# Autodesk Inventor assembly: 76607c01
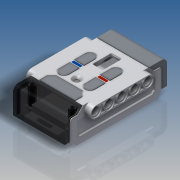
[picture p0: Inventor's stored thumbnail of the model, 180x180]
Saved by Autodesk Inventor 2016 SP2 (Build 200236200, 236)
## iProperties
Created: 2015-08-26
Part Number: 76607c01
Document SubType Name: Assembly
Designer: D. Kohfeld
Mass: 14.5113 g
Surface Area: 211.449 cm^2
Volume: 12.6712 cm^3
Density: 1.14522 g/cm^3
Author: D. Kohfeld
## Documents named in this file (8)
- A:\LEGO Pieces\EV3\76607c01.iam
- A:\LEGO Pieces\EV3\76607p01-White.ipt
- A:\LEGO Pieces\EV3\11235-TransBlackIRLens.ipt
- A:\LEGO Pieces\EV3\11235-LtBluishGray.ipt
- A:\LEGO Pieces\EV3\76608-White.ipt
- A:\LEGO Pieces\EV3\11236-LtBluishGray.ipt
- A:\LEGO Pieces\EV3\76610-LtBluishGray.ipt
- A:\LEGO Pieces\EV3\u9013-Black.ipt
## Components (13 placed, 7 different names)
1. 76607p01-White:1 — Mate:1, Mate:2, Mate:3, Mate:4, Flush:1, Flush:2, Flush:3, Flush:4, Angle:1, Angle:2, Angle:3, Angle:4, Mate:5, Flush:5, Flush:6, Mate:6, Flush:7, Mate:7, Flush:8, Flush:9, Mate:8, Angle:5
2. 11235-TransBlackIRLens:1 — Mate:6, Flush:7, Mate:7, Insert:1
3. 11235-LtBluishGray:1 — Flush:8, Flush:9, Mate:8
4. 76608-White:1 — Insert:1, Angle:5, Insert:2, Insert:3, Insert:4, Insert:5
5. 11236-LtBluishGray:1 — Mate:5, Flush:5, Flush:6
6. 76610-LtBluishGray:1 — Mate:1, Flush:3, Angle:2
7. 76610-LtBluishGray:2 — Mate:2, Flush:4, Angle:1
8. 76610-LtBluishGray:3 — Mate:3, Flush:2, Angle:4
9. 76610-LtBluishGray:4 — Mate:4, Flush:1, Angle:3
10. u9013-Black:1 — Insert:2
11. u9013-Black:2 — Insert:3
12. u9013-Black:3 — Insert:4
13. u9013-Black:4 — Insert:5
## Relationships (27: Flush 9, Mate 8, Angle 5, Insert 5)
- Mate:1: 76607p01-White:1 ↔ 76610-LtBluishGray:1
- Mate:2: 76607p01-White:1 ↔ 76610-LtBluishGray:2
- Mate:3: 76607p01-White:1 ↔ 76610-LtBluishGray:3
- Mate:4: 76607p01-White:1 ↔ 76610-LtBluishGray:4
- Flush:1: 76607p01-White:1 ↔ 76610-LtBluishGray:4
- Flush:2: 76607p01-White:1 ↔ 76610-LtBluishGray:3
- Flush:3: 76607p01-White:1 ↔ 76610-LtBluishGray:1
- Flush:4: 76607p01-White:1 ↔ 76610-LtBluishGray:2
- Angle:1 (0 deg): 76607p01-White:1 ↔ 76610-LtBluishGray:2
- Angle:2 (0 deg): 76607p01-White:1 ↔ 76610-LtBluishGray:1
- Angle:3 (0 deg): 76607p01-White:1 ↔ 76610-LtBluishGray:4
- Angle:4 (0 deg): 76607p01-White:1 ↔ 76610-LtBluishGray:3
- Mate:5: 76607p01-White:1 ↔ 11236-LtBluishGray:1
- Flush:5: 76607p01-White:1 ↔ 11236-LtBluishGray:1
- Flush:6: 76607p01-White:1 ↔ 11236-LtBluishGray:1
- Mate:6: 76607p01-White:1 ↔ 11235-TransBlackIRLens:1
- Flush:7: 76607p01-White:1 ↔ 11235-TransBlackIRLens:1
- Mate:7: 76607p01-White:1 ↔ 11235-TransBlackIRLens:1
- Flush:8: 76607p01-White:1 ↔ 11235-LtBluishGray:1
- Flush:9: 76607p01-White:1 ↔ 11235-LtBluishGray:1
- Mate:8: 76607p01-White:1 ↔ 11235-LtBluishGray:1
- Insert:1: 11235-TransBlackIRLens:1 ↔ 76608-White:1
- Angle:5 (0 deg): 76607p01-White:1 ↔ 76608-White:1
- Insert:2: 76608-White:1 ↔ u9013-Black:1
- Insert:3: 76608-White:1 ↔ u9013-Black:2
- Insert:4: 76608-White:1 ↔ u9013-Black:3
- Insert:5: 76608-White:1 ↔ u9013-Black:4
